# Autodesk Inventor assembly: Esteira-Y
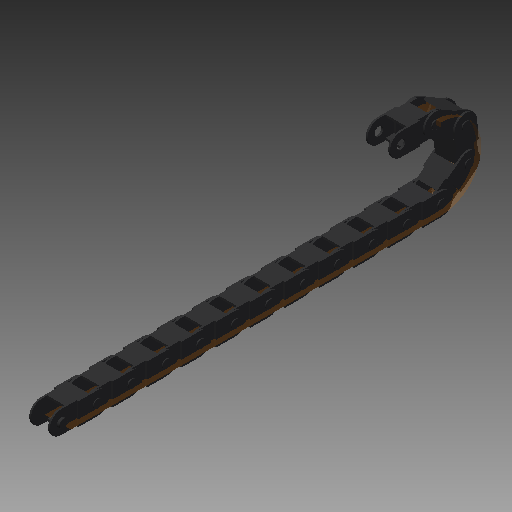
[picture p0: Inventor's stored thumbnail of the model, 512x512]
Saved by Autodesk Inventor 2017 (Build 210142000, 142)
## iProperties
Created: 2016-07-07
Part Number: Esteira-Y
Document SubType Name: Assembly
Designer: hmigu
Author: hmigu
## Documents named in this file (3)
- C:\Dropbox\Empresas\CNCBrasil\Projetos\Hardware\Mecânica\FDM\Office 600\Esteira-Y.iam
- C:\Dropbox\Empresas\CNCBrasil\Projetos\Hardware\Mecânica\Suprimentos\Eletrônica\Esteira-fesma-S10.ipt
- C:\Dropbox\Empresas\CNCBrasil\Projetos\Hardware\Mecânica\Suprimentos\Eletrônica\Esteira-fesma-S10-path-400.ipt
## Components (16 placed, 2 different names)
1. Esteira-fesma-S10-path-400:1 — Mate:19, Transitional:9, Mate:21, Transitional:10, Mate:23, Transitional:11, Mate:25, Transitional:12, Mate:27, Transitional:13, Mate:29, Transitional:14, Mate:31, Transitional:15, Mate:37, Angle:1, Mate:38, Mate:39, Transitional:16, Mate:41, Transitional:17, Angle:2, Mate:44, Transitional:19, Mate:46, Transitional:20, Tangent:1
2. Esteira-fesma-S10:5 — Mate:36, Mate:48
3. Esteira-fesma-S10:9 — Mate:19, Transitional:9, Mate:22, Mate:36
4. Esteira-fesma-S10:10 — Mate:21, Mate:22, Transitional:10, Mate:24
5. Esteira-fesma-S10:11 — Mate:23, Mate:24, Transitional:11, Mate:26
6. Esteira-fesma-S10:12 — Mate:25, Mate:26, Transitional:12, Mate:28
7. Esteira-fesma-S10:13 — Mate:27, Mate:28, Transitional:13, Mate:30
8. Esteira-fesma-S10:14 — Mate:29, Mate:30, Transitional:14, Mate:32
9. Esteira-fesma-S10:15 — Mate:31, Mate:32, Transitional:15, Mate:34, Mate:35
10. Esteira-fesma-S10:16 — Mate:37, Angle:1, Mate:38, Mate:52
11. Esteira-fesma-S10:17 — Mate:34, Mate:35, Flush:1, Tangent:1, Mate:53
12. Esteira-fesma-S10:18 — Mate:39, Transitional:16, Mate:42, Mate:52
13. Esteira-fesma-S10:19 — Mate:41, Mate:42, Transitional:17, Mate:45
14. Esteira-fesma-S10:20 — Flush:1, Angle:2, Mate:53
15. Esteira-fesma-S10:21 — Mate:44, Mate:45, Transitional:19, Mate:47
16. Esteira-fesma-S10:22 — Mate:46, Mate:47, Transitional:20, Mate:48
## Relationships (45: Mate 29, Transitional 12, Angle 2, Flush 1, Tangent 1)
- [Mate]: Esteira-fesma-S10-path-400:1 ↔ Esteira-fesma-S10:5
- [Transitional]: Esteira-fesma-S10-path-400:1 ↔ Esteira-fesma-S10:5
- Mate:19: Esteira-fesma-S10-path-400:1 ↔ Esteira-fesma-S10:9
- Transitional:9: Esteira-fesma-S10-path-400:1 ↔ Esteira-fesma-S10:9
- Mate:21: Esteira-fesma-S10-path-400:1 ↔ Esteira-fesma-S10:10
- Mate:22: Esteira-fesma-S10:9 ↔ Esteira-fesma-S10:10
- Transitional:10: Esteira-fesma-S10-path-400:1 ↔ Esteira-fesma-S10:10
- Mate:23: Esteira-fesma-S10-path-400:1 ↔ Esteira-fesma-S10:11
- Mate:24: Esteira-fesma-S10:10 ↔ Esteira-fesma-S10:11
- Transitional:11: Esteira-fesma-S10-path-400:1 ↔ Esteira-fesma-S10:11
- Mate:25: Esteira-fesma-S10-path-400:1 ↔ Esteira-fesma-S10:12
- Mate:26: Esteira-fesma-S10:11 ↔ Esteira-fesma-S10:12
- Transitional:12: Esteira-fesma-S10-path-400:1 ↔ Esteira-fesma-S10:12
- Mate:27: Esteira-fesma-S10-path-400:1 ↔ Esteira-fesma-S10:13
- Mate:28: Esteira-fesma-S10:12 ↔ Esteira-fesma-S10:13
- Transitional:13: Esteira-fesma-S10-path-400:1 ↔ Esteira-fesma-S10:13
- Mate:29: Esteira-fesma-S10-path-400:1 ↔ Esteira-fesma-S10:14
- Mate:30: Esteira-fesma-S10:13 ↔ Esteira-fesma-S10:14
- Transitional:14: Esteira-fesma-S10-path-400:1 ↔ Esteira-fesma-S10:14
- Mate:31: Esteira-fesma-S10-path-400:1 ↔ Esteira-fesma-S10:15
- Mate:32: Esteira-fesma-S10:14 ↔ Esteira-fesma-S10:15
- Transitional:15: Esteira-fesma-S10-path-400:1 ↔ Esteira-fesma-S10:15
- Mate:34: Esteira-fesma-S10:15 ↔ Esteira-fesma-S10:17
- Mate:35: Esteira-fesma-S10:15 ↔ Esteira-fesma-S10:17
- Mate:36: Esteira-fesma-S10:5 ↔ Esteira-fesma-S10:9
- Mate:37: Esteira-fesma-S10-path-400:1 ↔ Esteira-fesma-S10:16
- Angle:1 (0 deg): Esteira-fesma-S10-path-400:1 ↔ Esteira-fesma-S10:16
- Mate:38: Esteira-fesma-S10-path-400:1 ↔ Esteira-fesma-S10:16
- Mate:39: Esteira-fesma-S10-path-400:1 ↔ Esteira-fesma-S10:18
- Transitional:16: Esteira-fesma-S10-path-400:1 ↔ Esteira-fesma-S10:18
- Mate:41: Esteira-fesma-S10-path-400:1 ↔ Esteira-fesma-S10:19
- Mate:42: Esteira-fesma-S10:18 ↔ Esteira-fesma-S10:19
- Transitional:17: Esteira-fesma-S10-path-400:1 ↔ Esteira-fesma-S10:19
- Flush:1: Esteira-fesma-S10:17 ↔ Esteira-fesma-S10:20
- Angle:2 (0 deg): Esteira-fesma-S10-path-400:1 ↔ Esteira-fesma-S10:20
- Mate:44: Esteira-fesma-S10-path-400:1 ↔ Esteira-fesma-S10:21
- Mate:45: Esteira-fesma-S10:19 ↔ Esteira-fesma-S10:21
- Transitional:19: Esteira-fesma-S10-path-400:1 ↔ Esteira-fesma-S10:21
- Mate:46: Esteira-fesma-S10-path-400:1 ↔ Esteira-fesma-S10:22
- Mate:47: Esteira-fesma-S10:21 ↔ Esteira-fesma-S10:22
- Transitional:20: Esteira-fesma-S10-path-400:1 ↔ Esteira-fesma-S10:22
- Mate:48: Esteira-fesma-S10:5 ↔ Esteira-fesma-S10:22
- Tangent:1: Esteira-fesma-S10-path-400:1 ↔ Esteira-fesma-S10:17
- Mate:52: Esteira-fesma-S10:16 ↔ Esteira-fesma-S10:18
- Mate:53: Esteira-fesma-S10:17 ↔ Esteira-fesma-S10:20
